# Autodesk Inventor assembly: videotest1
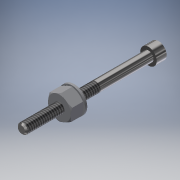
[picture p0: Inventor's stored thumbnail of the model, 180x180]
Saved by Autodesk Inventor 2017 (Build 210142000, 142)
## iProperties
Created: 2018-03-21
Part Number: videotest1
Document SubType Name: Assembly
Designer: User
Author: User
## Documents named in this file (3)
- C:\Robotics\CAD\2018-19_CAD\Offseason\videotest1.iam
- C:\Robotics\CAD\COTSParts\Fasteners\6-32 locknut.ipt
- C:\Robotics\CAD\COTSParts\Fasteners\6-32 SHCS x1750.ipt
## Components (2 placed, 2 different names)
1. 6-32 locknut:1 — Mate:1
2. 6-32 SHCS x1750:1 — Mate:1
## Relationships (1: Mate 1)
- Mate:1: 6-32 locknut:1 ↔ 6-32 SHCS x1750:1
